# Autodesk Inventor assembly: Arm for Gen 2
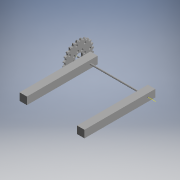
[picture p0: Inventor's stored thumbnail of the model, 180x180]
Saved by Autodesk Inventor 2019 (Build 230136000, 136)
## iProperties
Part Number: Arm for Gen 2
Document SubType Name: Assembly
Designer: Delta
Author: Delta
## Documents named in this file (4)
- C:\Robotics\2019-20_CAD\Collection\Arm for Gen 2.iam
- C:\Robotics\2019-20_CAD\Collection\30x30 pillars.ipt
- C:\Robotics\2019-20_CAD\Collection\12 Inch Hex Axle.ipt
- C:\Robotics\COTSParts\Sprockets - AndyMark\615106.ipt
## Components (4 placed, 3 different names)
1. 30x30 pillars:1 — Mate:1, Flush:1, Mate:2, Flush:2, Mate:4
2. 30x30 pillars:2 — Mate:3, Flush:2, Mate:4
3. 12 Inch Hex Axle:1 — Mate:1, Flush:1, Mate:2, Mate:3, Mate:5, Flush:3
4. 615106:1 — Mate:5, Flush:3
## Relationships (8: Mate 5, Flush 3)
- Mate:1: 30x30 pillars:1 ↔ 12 Inch Hex Axle:1
- Flush:1: 30x30 pillars:1 ↔ 12 Inch Hex Axle:1
- Mate:2: 30x30 pillars:1 ↔ 12 Inch Hex Axle:1
- Mate:3: 30x30 pillars:2 ↔ 12 Inch Hex Axle:1
- Flush:2: 30x30 pillars:1 ↔ 30x30 pillars:2
- Mate:4 (85 mm): 30x30 pillars:1 ↔ 30x30 pillars:2
- Mate:5: 12 Inch Hex Axle:1 ↔ 615106:1
- Flush:3: 12 Inch Hex Axle:1 ↔ 615106:1
